# Autodesk Inventor assembly: motor_base
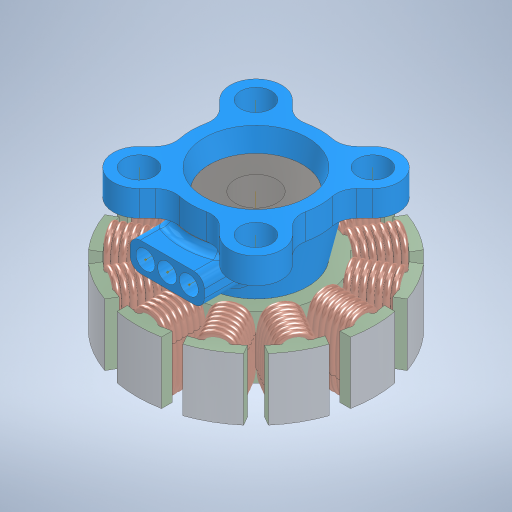
[picture p0: Inventor's stored thumbnail of the model, 512x512]
Saved by Autodesk Inventor 2024 (Build 280153000, 153)
## iProperties
Created: 2024-03-08
Part Number: motor_base
Document SubType Name: Assembly
Designer: nicoe
Mass: 19.4806 g
Surface Area: 69.0526 cm^2
Volume: 2.4816 cm^3
Density: 7.85 g/cm^3
Sending System: Creo  TM  7.0
Author: nicoe
## Documents named in this file (6)
- D:\users\nicoe\OneDrive\OneDrive - Stellenbosch University\Desktop\Nico_Masters\1. Drone Constrution\CAD Files\iflight xing-e 2306(To replace R5)\Broken up motor\motor_base.iam
- D:\users\nicoe\OneDrive\OneDrive - Stellenbosch University\Desktop\Nico_Masters\1. Drone Constrution\CAD Files\iflight xing-e 2306(To replace R5)\motor xing\cely_motor\MOTOR_GUMICKA.ipt
- D:\users\nicoe\OneDrive\OneDrive - Stellenbosch University\Desktop\Nico_Masters\1. Drone Constrution\CAD Files\iflight xing-e 2306(To replace R5)\motor xing\cely_motor\MOTOR_PODLOZKA.ipt
- D:\users\nicoe\OneDrive\OneDrive - Stellenbosch University\Desktop\Nico_Masters\1. Drone Constrution\CAD Files\iflight xing-e 2306(To replace R5)\motor xing\cely_motor\MOTOR_SPODOK.ipt
- D:\users\nicoe\OneDrive\OneDrive - Stellenbosch University\Desktop\Nico_Masters\1. Drone Constrution\CAD Files\iflight xing-e 2306(To replace R5)\motor xing\cely_motor\MOTOR_SPODOK_1.ipt
- D:\users\nicoe\OneDrive\OneDrive - Stellenbosch University\Desktop\Nico_Masters\1. Drone Constrution\CAD Files\iflight xing-e 2306(To replace R5)\Broken up motor\BearingReplacement.ipt
## Components (6 placed, 5 different names)
1. MOTOR_GUMICKA
2. MOTOR_PODLOZKA
3. MOTOR_SPODOK — Mate:1, Mate:2, Mate:4, Mate:5
4. MOTOR_SPODOK_1
5. BearingReplacement:1 — Mate:1, Mate:2, Mate:3
6. BearingReplacement:2 — Mate:4, Mate:5, Mate:6
## Relationships (6: Mate 6)
- Mate:1: MOTOR_SPODOK ↔ BearingReplacement:1
- Mate:2: MOTOR_SPODOK ↔ BearingReplacement:1
- Mate:3: BearingReplacement:1
- Mate:4: MOTOR_SPODOK ↔ BearingReplacement:2
- Mate:5: MOTOR_SPODOK ↔ BearingReplacement:2
- Mate:6: BearingReplacement:2
